# Autodesk Inventor assembly: Assembly
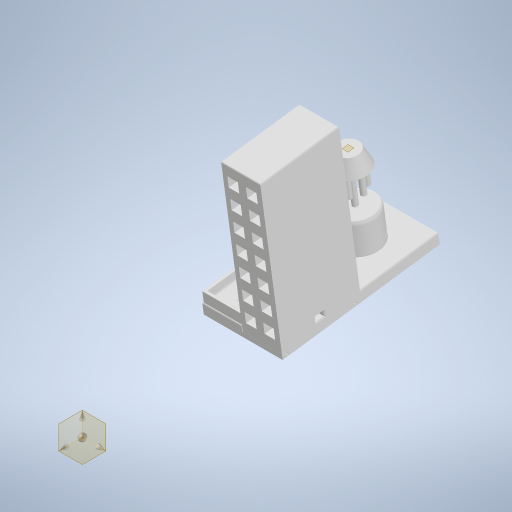
[picture p0: Inventor's stored thumbnail of the model, 512x512]
Saved by Autodesk Inventor 2024.3 (Build 283343000, 343)
## iProperties
Created: 2024-08-06
Part Number: Assembly
Document SubType Name: Assembly
Designer: lordk
Author: lordk
## Documents named in this file (6)
- C:\Users\lordk\Github\ROBIT_Intern_KiHongPark_HW_repo\Projects\HW_Design\HomeWork\HW_20240806\19th_KihongPark_04\Assembly.iam
- C:\Users\lordk\Github\ROBIT_Intern_KiHongPark_HW_repo\Projects\HW_Design\HomeWork\HW_20240806\19th_KihongPark_04\Body.ipt
- C:\Users\lordk\Github\ROBIT_Intern_KiHongPark_HW_repo\Projects\HW_Design\HomeWork\HW_20240806\19th_KihongPark_04\Control_Tower.ipt
- C:\Users\lordk\Github\ROBIT_Intern_KiHongPark_HW_repo\Projects\HW_Design\HomeWork\HW_20240806\19th_KihongPark_04\Small_Tower.ipt
- C:\Users\lordk\Github\ROBIT_Intern_KiHongPark_HW_repo\Projects\HW_Design\HomeWork\HW_20240806\19th_KihongPark_04\Small_Tower2.ipt
- C:\Users\lordk\Github\ROBIT_Intern_KiHongPark_HW_repo\Projects\HW_Design\HomeWork\HW_20240806\19th_KihongPark_04\Main_Tower.ipt
## Components (5 placed, 5 different names)
1. Body:1 — Mate:2, Mate:3, Mate:4, Mate:5, Mate:6, Mate:7, Mate:8, Mate:9, Mate:10, Mate:11
2. Control_Tower:1 — Mate:2, Mate:3, Mate:4
3. Small_Tower:1 — Mate:5, Mate:6, Mate:7
4. Small_Tower2:1 — Mate:8, Mate:9
5. Main_Tower:1 — Mate:10, Mate:11
## Relationships (10: Mate 10)
- Mate:2: Body:1 ↔ Control_Tower:1
- Mate:3: Body:1 ↔ Control_Tower:1
- Mate:4: Body:1 ↔ Control_Tower:1
- Mate:5: Body:1 ↔ Small_Tower:1
- Mate:6: Body:1 ↔ Small_Tower:1
- Mate:7: Body:1 ↔ Small_Tower:1
- Mate:8: Body:1 ↔ Small_Tower2:1
- Mate:9: Body:1 ↔ Small_Tower2:1
- Mate:10: Body:1 ↔ Main_Tower:1
- Mate:11: Body:1 ↔ Main_Tower:1
